# Autodesk Inventor assembly: ГЛАЗ НОВЫЙ СБОРКА_ЗЕРКАЛО
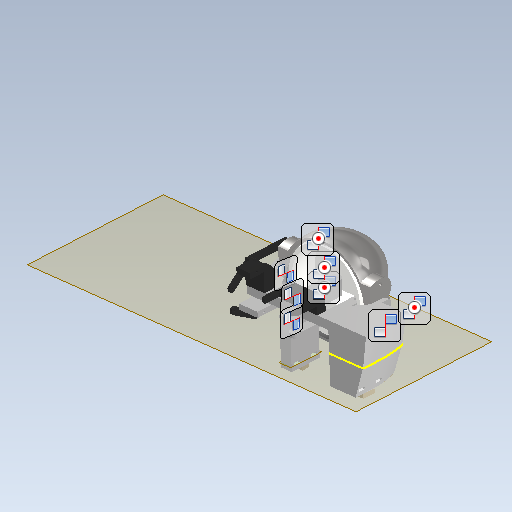
[picture p0: Inventor's stored thumbnail of the model, 512x512]
Saved by Autodesk Inventor 2020 (Build 240168000, 168)
## iProperties
Created: 2022-02-16
Part Number: ГЛАЗ НОВЫЙ СБОРКА_ЗЕРКАЛО
Document SubType Name: Assembly
Designer: Администратор
Author: Администратор
## Documents named in this file (11)
- H:\OnStage\face_cborka\Лицо_пересборка\Глаз\Face 2.0 full\ГЛАЗ НОВЫЙ СБОРКА_ЗЕРКАЛО.iam
- H:\OnStage\face_cborka\Лицо_пересборка\Глаз\Face 2.0 full\шатун движенияглаза_ЗЕРКАЛО.ipt
- H:\OnStage\face_cborka\Лицо_пересборка\Глаз\Face 2.0 full\нижнее веко_ЗЕРКАЛО.ipt
- H:\OnStage\face_cborka\Лицо_пересборка\Глаз\Face 2.0 full\держалка сервы движения глаз_ЗЕРКАЛО.ipt
- H:\OnStage\face_cborka\Лицо_пересборка\Глаз\Face 2.0 full\держалка сервы век_ЗЕРКАЛО.ipt
- H:\OnStage\face_cborka\Лицо_пересборка\Глаз\Face 2.0 full\держалка глаза_ЗЕРКАЛО.ipt
- H:\OnStage\face_cborka\Лицо_пересборка\Глаз\Face 2.0 full\верхнее веко_ЗЕРКАЛО.ipt
- H:\OnStage\face_cborka\Лицо_пересборка\Глаз\Face 2.0 full\нижний шатун век_ЗЕРКАЛО.ipt
- H:\OnStage\face_cborka\Лицо_пересборка\Глаз\Face 2.0 full\зрачок_ЗЕРКАЛО.ipt
- H:\OnStage\face_cborka\Лицо_пересборка\Глаз\Face 2.0 full\белок глаза_ЗЕРКАЛО_ЗЕРКАЛО.ipt
- H:\OnStage\face_cborka\Лицо_пересборка\Глаз\Face 2.0 full\верхний шатун века_ЗЕРКАЛО1_ЗЕРКАЛО.ipt
## Components (10 placed, 10 different names)
1. шатун движенияглаза_ЗЕРКАЛО:1 — Совмещение:47, Совмещение:46
2. нижнее веко_ЗЕРКАЛО:1 — Совмещение:7, Совмещение:6, Совмещение:42, Совмещение:41, Совмещение:36, Угол:1
3. держалка сервы движения глаз_ЗЕРКАЛО:1 — Совмещение:34, Совмещение:33, Совмещение:32
4. держалка сервы век_ЗЕРКАЛО:1
5. держалка глаза_ЗЕРКАЛО:1 — Совмещение:34, Совмещение:33, Совмещение:32, Совмещение:7, Совмещение:6, Совмещение:48, Совмещение:45, Угол:3
6. верхний шатун века_ЗЕРКАЛО1_ЗЕРКАЛО:1 — Совмещение:42, Совмещение:41, Угол:3
7. верхнее веко_ЗЕРКАЛО:1 — Совмещение:14, Совмещение:13, Совмещение:35, Совмещение:36, Угол:2
8. нижний шатун век_ЗЕРКАЛО:1 — Совмещение:14, Совмещение:13
9. зрачок_ЗЕРКАЛО:1 — Совмещение:40, Совмещение:39
10. белок глаза_ЗЕРКАЛО_ЗЕРКАЛО:1 — Совмещение:48, Совмещение:47, Совмещение:46, Совмещение:45, Совмещение:40, Совмещение:39, Совмещение:35, Угол:1, Угол:2
## Relationships (20: Mate 17, Angle 3)
- Совмещение:34 [Mate]: держалка сервы движения глаз_ЗЕРКАЛО:1 ↔ держалка глаза_ЗЕРКАЛО:1
- Совмещение:33 [Mate]: держалка сервы движения глаз_ЗЕРКАЛО:1 ↔ держалка глаза_ЗЕРКАЛО:1
- Совмещение:32 [Mate]: держалка сервы движения глаз_ЗЕРКАЛО:1 ↔ держалка глаза_ЗЕРКАЛО:1
- Совмещение:7 [Mate]: нижнее веко_ЗЕРКАЛО:1 ↔ держалка глаза_ЗЕРКАЛО:1
- Совмещение:6 [Mate]: нижнее веко_ЗЕРКАЛО:1 ↔ держалка глаза_ЗЕРКАЛО:1
- Совмещение:14 [Mate]: верхнее веко_ЗЕРКАЛО:1 ↔ нижний шатун век_ЗЕРКАЛО:1
- Совмещение:13 [Mate]: верхнее веко_ЗЕРКАЛО:1 ↔ нижний шатун век_ЗЕРКАЛО:1
- Совмещение:48 [Mate]: держалка глаза_ЗЕРКАЛО:1 ↔ белок глаза_ЗЕРКАЛО_ЗЕРКАЛО:1
- Совмещение:47 [Mate]: шатун движенияглаза_ЗЕРКАЛО:1 ↔ белок глаза_ЗЕРКАЛО_ЗЕРКАЛО:1
- Совмещение:46 [Mate]: шатун движенияглаза_ЗЕРКАЛО:1 ↔ белок глаза_ЗЕРКАЛО_ЗЕРКАЛО:1
- Совмещение:45 [Mate]: держалка глаза_ЗЕРКАЛО:1 ↔ белок глаза_ЗЕРКАЛО_ЗЕРКАЛО:1
- Совмещение:40 [Mate]: зрачок_ЗЕРКАЛО:1 ↔ белок глаза_ЗЕРКАЛО_ЗЕРКАЛО:1
- Совмещение:39 [Mate]: зрачок_ЗЕРКАЛО:1 ↔ белок глаза_ЗЕРКАЛО_ЗЕРКАЛО:1
- Совмещение:42 [Mate]: нижнее веко_ЗЕРКАЛО:1 ↔ верхний шатун века_ЗЕРКАЛО1_ЗЕРКАЛО:1
- Совмещение:41 [Mate]: нижнее веко_ЗЕРКАЛО:1 ↔ верхний шатун века_ЗЕРКАЛО1_ЗЕРКАЛО:1
- Совмещение:35 [Mate]: верхнее веко_ЗЕРКАЛО:1 ↔ белок глаза_ЗЕРКАЛО_ЗЕРКАЛО:1
- Совмещение:36 [Mate]: нижнее веко_ЗЕРКАЛО:1 ↔ верхнее веко_ЗЕРКАЛО:1
- Угол:1 [Angle] (0 deg): нижнее веко_ЗЕРКАЛО:1 ↔ белок глаза_ЗЕРКАЛО_ЗЕРКАЛО:1
- Угол:2 [Angle] (0 deg): верхнее веко_ЗЕРКАЛО:1 ↔ белок глаза_ЗЕРКАЛО_ЗЕРКАЛО:1
- Угол:3 [Angle] (0 deg): держалка глаза_ЗЕРКАЛО:1 ↔ верхний шатун века_ЗЕРКАЛО1_ЗЕРКАЛО:1
